# Autodesk Inventor assembly: subflap2
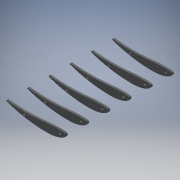
[picture p0: Inventor's stored thumbnail of the model, 180x180]
Saved by Autodesk Inventor 2018 (Build 220112000, 112)
## iProperties
Created: 2018-03-05
Part Number: subflap2
Material: 一般
Document SubType Name: Assembly
Designer: ku_sk
Author: ku_sk
## Documents named in this file (2)
- D:\Users\ku_sk\Documents\Inventor\Aero\KS-15\Fr.wing\parts\subflap\subflap.iam
- D:\Users\ku_sk\Documents\Inventor\Aero\KS-15\Fr.wing\parts\subflap\plate_sf.ipt
## Components (6 placed, 1 different names)
1. plate_sf:1 — メイト:1, メイト:2, メイト:3, メイト:4, フラッシュ:2, メイト:5, メイト:14
2. plate_sf:2 — フラッシュ:1, メイト:2, メイト:3, メイト:9, メイト:10
3. plate_sf:3 — フラッシュ:2, フラッシュ:3, メイト:5, メイト:6, メイト:13, メイト:14
4. plate_sf:4 — フラッシュ:3, フラッシュ:4, メイト:6, メイト:7, メイト:12, メイト:13
5. plate_sf:5 — フラッシュ:4, フラッシュ:5, メイト:7, メイト:8, メイト:11, メイト:12
6. plate_sf:6 — フラッシュ:5, メイト:8, メイト:9, メイト:10, メイト:11
## Relationships (19: Mate 14, Flush 5)
- メイト:1 [Mate] (-110 mm): plate_sf:1
- フラッシュ:1 [Flush] (-115 mm): plate_sf:2
- メイト:2 [Mate]: plate_sf:1 ↔ plate_sf:2
- メイト:3 [Mate]: plate_sf:1 ↔ plate_sf:2
- メイト:4 [Mate]: plate_sf:1
- フラッシュ:2 [Flush] (-44.2 mm): plate_sf:1 ↔ plate_sf:3
- フラッシュ:3 [Flush] (-44.2 mm): plate_sf:3 ↔ plate_sf:4
- フラッシュ:4 [Flush] (-44.2 mm): plate_sf:4 ↔ plate_sf:5
- フラッシュ:5 [Flush] (-44.2 mm): plate_sf:5 ↔ plate_sf:6
- メイト:5 [Mate]: plate_sf:1 ↔ plate_sf:3
- メイト:6 [Mate]: plate_sf:3 ↔ plate_sf:4
- メイト:7 [Mate]: plate_sf:4 ↔ plate_sf:5
- メイト:8 [Mate]: plate_sf:5 ↔ plate_sf:6
- メイト:9 [Mate]: plate_sf:2 ↔ plate_sf:6
- メイト:10 [Mate]: plate_sf:2 ↔ plate_sf:6
- メイト:11 [Mate]: plate_sf:5 ↔ plate_sf:6
- メイト:12 [Mate]: plate_sf:4 ↔ plate_sf:5
- メイト:13 [Mate]: plate_sf:3 ↔ plate_sf:4
- メイト:14 [Mate]: plate_sf:1 ↔ plate_sf:3
